# Autodesk Inventor assembly: CL7-100
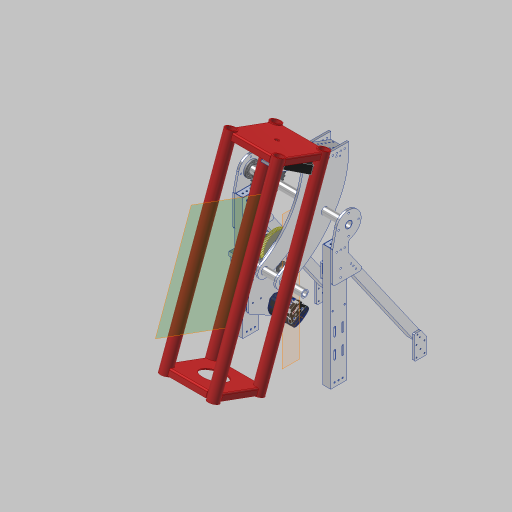
[picture p0: Inventor's stored thumbnail of the model, 512x512]
Saved by Autodesk Inventor 2023.5 (Build 275446000, 446)
## iProperties
Created: 2025-03-17
Part Number: CL7-100
Document SubType Name: Assembly
Designer: dlangdon
Author: dlangdon
## Documents named in this file (16)
- C:\Users\slick\OneDrive\Desktop\2025-ReefScape---CAD\Climber\CL7\CL7-100.iam
- C:\Users\slick\OneDrive\Desktop\2025-ReefScape---CAD\Climber\CL7\CL7-001.ipt
- C:\Users\slick\OneDrive\Desktop\2025-ReefScape---CAD\Climber\CL7\CL-002.ipt
- C:\Users\slick\OneDrive\Desktop\2025-ReefScape---CAD\Climber\CL7\CL7-003.ipt
- C:\Users\slick\OneDrive\Desktop\2025-ReefScape---CAD\COMMON PARTS\BEARINGS\0_875_ID_1_875OD_0_375_Thick60355K508_Ball Bearing.ipt
- C:\Users\slick\OneDrive\Desktop\2025-ReefScape---CAD\Elevator\EL2\EL2-005.ipt
- C:\Users\slick\OneDrive\Desktop\2025-ReefScape---CAD\Climber\CL7\CL7-200.iam
- C:\Users\slick\OneDrive\Desktop\2025-ReefScape---CAD\Field Items\Full Field\FE-2025\GE-25201.iam
- C:\Users\slick\OneDrive\Desktop\2025-ReefScape---CAD\Climber\CL7\CL7-010.ipt
- C:\Users\slick\OneDrive\Desktop\2025-ReefScape---CAD\Climber\CL7\CL7-010_MIR.ipt
- C:\Users\slick\OneDrive\Desktop\2025-ReefScape---CAD\Climber\CL7\CL7-012.ipt
- C:\Users\slick\OneDrive\Desktop\2025-ReefScape---CAD\Climber\CL7\CL7-011.ipt
- C:\Users\slick\OneDrive\Desktop\2025-ReefScape---CAD\Climber\CL7\CL-GB\CL7-GB-100.iam
- C:\Users\slick\OneDrive\Desktop\2025-ReefScape---CAD\Climber\CL7\CL7-014.ipt
- C:\Users\slick\OneDrive\Desktop\2025-ReefScape---CAD\COMMON PARTS\SPROCKETS\35\36t_Aluminum_Plate_Sprocket_35_Chain_1-1_8_Bearing_Bore_217-2649.ipt
- C:\Users\slick\OneDrive\Desktop\2025-ReefScape---CAD\Climber\CL7\CL-GB\CL7-GB-005.ipt
## Components (23 placed, 15 different names)
1. CL7-001:1 — Flush:1, Flush:2, Mate:1, Insert:3, Insert:4, Insert:7, Insert:8, Symmetry:2, Mate:7, Flush:3, Flush:6, Insert:9, Insert:10, Insert:20, Insert:21, Insert:22, Insert:23
2. CL7-001:2 — Flush:1, Flush:2, Mate:1, Insert:1, Insert:2, Insert:5, Insert:6, Symmetry:2, Flush:5, Mate:8, Insert:11, Insert:12, Insert:18
3. CL-002:1 — Mate:7, Flush:3, Flush:4, Flush:6, Insert:13, Insert:14, Insert:17
4. CL-002:2 — Flush:4, Flush:5, Mate:8, Insert:15, Insert:16, Insert:19
5. CL7-003:1 — Mate:4, Mate:5, Mate:6, Mate:14, Mate:17, Mate:18
6. 0_875_ID_1_875OD_0_375_Thick60355K508_Ball Bearing:1 — Mate:4, Symmetry:1, Mate:16
7. 0_875_ID_1_875OD_0_375_Thick60355K508_Ball Bearing:2 — Mate:5, Symmetry:1, Mate:15
8. EL2-005:1 — Insert:1, Insert:2
9. EL2-005:2 — Insert:3, Insert:4
10. EL2-005:3 — Insert:5, Insert:6
11. EL2-005:4 — Insert:7, Insert:8
12. CL7-010:1 — Insert:9, Insert:10, Mate:16
13. CL7-200:1 [sub-assembly] — Mate:6, Mate:9, Mate:10, Mate:11, Mate:12, Mate:13
14. GE-25201:1 [sub-assembly] — Mate:10, Mate:11, Mate:12, Mate:13
15. CL7-010_MIR:1 — Mate:14, Mate:15, Insert:11, Insert:12
16. CL7-012:1 — Insert:13, Insert:14
17. CL7-012:2 — Insert:15, Insert:16
18. CL7-011:1 — Insert:17
19. CL7-011:2 — Insert:18, Insert:19
20. CL7-GB-100:1 [sub-assembly] — Insert:20, Insert:21, Flush:7
21. CL7-014:1 — Insert:22, Insert:23
22. 36t_Aluminum_Plate_Sprocket_35_Chain_1-1_8_Bearing_Bore_217-2649:1 — Mate:17, Flush:7, Insert:24
23. CL7-GB-005:1 — Mate:18, Insert:24
## Relationships (49: Insert 24, Mate 16, Flush 7, Symmetry 2)
- Flush:1: CL7-001:1 ↔ CL7-001:2
- Flush:2: CL7-001:1 ↔ CL7-001:2
- Mate:1 (254 mm): CL7-001:1 ↔ CL7-001:2
- Mate:4: CL7-003:1 ↔ 0_875_ID_1_875OD_0_375_Thick60355K508_Ball Bearing:1
- Mate:5: CL7-003:1 ↔ 0_875_ID_1_875OD_0_375_Thick60355K508_Ball Bearing:2
- Symmetry:1: 0_875_ID_1_875OD_0_375_Thick60355K508_Ball Bearing:1 ↔ 0_875_ID_1_875OD_0_375_Thick60355K508_Ball Bearing:2
- Insert:1: CL7-001:2 ↔ EL2-005:1
- Insert:2: CL7-001:2 ↔ EL2-005:1
- Insert:3: CL7-001:1 ↔ EL2-005:2
- Insert:4: CL7-001:1 ↔ EL2-005:2
- Insert:5: CL7-001:2 ↔ EL2-005:3
- Insert:6: CL7-001:2 ↔ EL2-005:3
- Insert:7: CL7-001:1 ↔ EL2-005:4
- Insert:8: CL7-001:1 ↔ EL2-005:4
- Mate:6: CL7-003:1 ↔ CL7-200:1
- Symmetry:2: CL7-001:1 ↔ CL7-001:2
- Mate:7: CL7-001:1 ↔ CL-002:1
- Flush:3: CL7-001:1 ↔ CL-002:1
- Flush:4: CL-002:1 ↔ CL-002:2
- Flush:5: CL7-001:2 ↔ CL-002:2
- Mate:8: CL7-001:2 ↔ CL-002:2
- Flush:6: CL7-001:1 ↔ CL-002:1
- Mate:9 (50.8 mm): CL7-200:1
- Mate:10: CL7-200:1 ↔ GE-25201:1
- Mate:11: CL7-200:1 ↔ GE-25201:1
- Mate:12: CL7-200:1 ↔ GE-25201:1
- Mate:13 (25.4 mm): CL7-200:1 ↔ GE-25201:1
- Insert:9: CL7-001:1 ↔ CL7-010:1
- Insert:10: CL7-001:1 ↔ CL7-010:1
- Mate:14: CL7-003:1 ↔ CL7-010_MIR:1
- Mate:15: 0_875_ID_1_875OD_0_375_Thick60355K508_Ball Bearing:2 ↔ CL7-010_MIR:1
- Insert:11: CL7-001:2 ↔ CL7-010_MIR:1
- Insert:12: CL7-001:2 ↔ CL7-010_MIR:1
- Mate:16: 0_875_ID_1_875OD_0_375_Thick60355K508_Ball Bearing:1 ↔ CL7-010:1
- Insert:13: CL-002:1 ↔ CL7-012:1
- Insert:14: CL-002:1 ↔ CL7-012:1
- Insert:15: CL-002:2 ↔ CL7-012:2
- Insert:16: CL-002:2 ↔ CL7-012:2
- Insert:17: CL-002:1 ↔ CL7-011:1
- Insert:18: CL7-001:2 ↔ CL7-011:2
- Insert:19: CL-002:2 ↔ CL7-011:2
- Insert:20: CL7-001:1 ↔ CL7-GB-100:1
- Insert:21: CL7-001:1 ↔ CL7-GB-100:1
- Insert:22: CL7-001:1 ↔ CL7-014:1
- Insert:23: CL7-001:1 ↔ CL7-014:1
- Mate:17: CL7-003:1 ↔ 36t_Aluminum_Plate_Sprocket_35_Chain_1-1_8_Bearing_Bore_217-2649:1
- Flush:7: CL7-GB-100:1 ↔ 36t_Aluminum_Plate_Sprocket_35_Chain_1-1_8_Bearing_Bore_217-2649:1
- Mate:18: CL7-003:1 ↔ CL7-GB-005:1
- Insert:24: 36t_Aluminum_Plate_Sprocket_35_Chain_1-1_8_Bearing_Bore_217-2649:1 ↔ CL7-GB-005:1
